# Autodesk Inventor assembly: m3X16
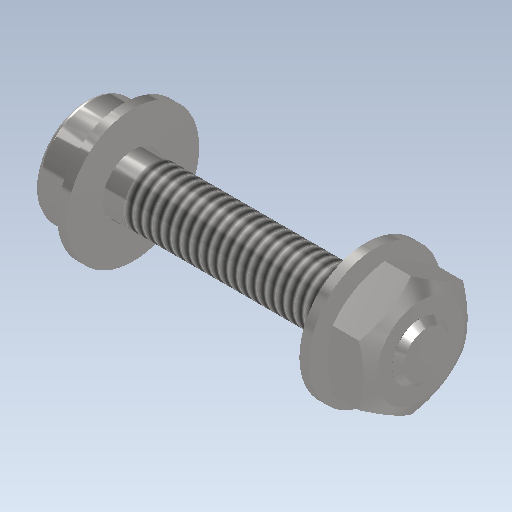
[picture p0: Inventor's stored thumbnail of the model, 512x512]
Saved by Autodesk Inventor 2020 (Build 240168000, 168)
## iProperties
Created: 2021-02-25
Part Number: m3X16
Document SubType Name: Assembly
Designer: Iulian Bors
Mass: 1.81981 g
Surface Area: 4.88857 cm^2
Volume: 0.231823 cm^3
Density: 7.85 g/cm^3
Author: Iulian Bors
## Documents named in this file (4)
- Z:\I.A.B\Proiecte\0008 I.A.B 3D 2.1 Imprimanta aracet Metal\10 Mecanic\m3X16.iam
- Z:\I.A.B\Proiecte\0008 I.A.B 3D 2.1 Imprimanta aracet Metal\10 Mecanic\0008-10-2005 DIN 125 - A 3.2.ipt
- Z:\I.A.B\Proiecte\0008 I.A.B 3D 2.1 Imprimanta aracet Metal\10 Mecanic\0008-10-2006 DIN 7984 - M3 x 16.ipt
- Z:\I.A.B\Proiecte\0008 I.A.B 3D 2.1 Imprimanta aracet Metal\10 Mecanic\0008-10-2009 DIN 555-5 - M3.ipt
## Components (4 placed, 3 different names)
1. 0008-10-2006 DIN 7984 - M3 x 16.ipt:1 — Insert:1, Insert:2
2. 0008-10-2009 DIN 555-5 - M3.ipt:2 — Insert:1, Insert:3
3. 0008-10-2005 DIN 125 - A 3.2.ipt:3 — Insert:2
4. 0008-10-2005 DIN 125 - A 3.2.ipt:4 — Insert:3
## Relationships (3: Insert 3)
- Insert:1: 0008-10-2006 DIN 7984 - M3 x 16.ipt:1 ↔ 0008-10-2009 DIN 555-5 - M3.ipt:2
- Insert:2: 0008-10-2006 DIN 7984 - M3 x 16.ipt:1 ↔ 0008-10-2005 DIN 125 - A 3.2.ipt:3
- Insert:3: 0008-10-2009 DIN 555-5 - M3.ipt:2 ↔ 0008-10-2005 DIN 125 - A 3.2.ipt:4
